# Autodesk Inventor assembly: ontel_installed
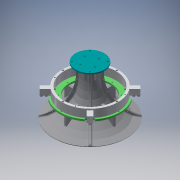
[picture p0: Inventor's stored thumbnail of the model, 180x180]
Saved by Autodesk Inventor 2016 (Build 200138000, 138)
## iProperties
Created: 2015-12-11
Part Number: ontel_installed
Document SubType Name: Assembly
Designer: ddeboer
Author: ddeboer
## Documents named in this file (5)
- C:\Users\Dave\Desktop\leuschner-cad\ontel_installed.iam
- C:\Users\Dave\Desktop\leuschner-cad\onTelMountingAssy.iam
- C:\Users\Dave\Desktop\leuschner-cad\Quad Assy.iam
- C:\Users\Dave\Desktop\leuschner-cad\cover.ipt
- C:\Users\Dave\Desktop\leuschner-cad\qtr20_175.ipt
## Components (7 placed, 4 different names)
1. onTelMountingAssy:1 [sub-assembly] — Insert:7, Insert:10
2. Quad Assy:1 [sub-assembly]
3. cover:1 — Insert:7
4. qtr20_175:1 — Insert:10
5. qtr20_175:2
6. qtr20_175:3
7. qtr20_175:4
## Component patterns: (4 elements, first: qtr20_175:1)
## Relationships (2: Insert 2)
- Insert:7 (-12.7 mm): onTelMountingAssy:1 ↔ cover:1
- Insert:10: onTelMountingAssy:1 ↔ qtr20_175:1
